# Autodesk Inventor assembly: electromag_gimbal
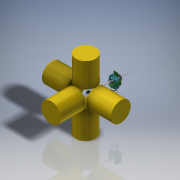
[picture p0: Inventor's stored thumbnail of the model, 180x180]
Saved by Autodesk Inventor 2019 (Build 230136000, 136)
## iProperties
Created: 2018-08-27
Part Number: electromag_gimbal
Document SubType Name: Assembly
Designer: Brian
Author: Brian
## Documents named in this file (13)
- C:\Users\Brian\Desktop\designs\gimbal\electromag_gimbal.iam
- C:\Users\Brian\Desktop\designs\gimbal\aluminum rod.ipt
- C:\Users\Brian\Desktop\designs\gimbal\61205K720_FIXED ALIGNMENT LINEAR BALL BRNG.ipt
- C:\Users\Brian\Desktop\designs\gimbal\magnet.ipt
- C:\Users\Brian\Desktop\designs\gimbal\angle hall sensor.ipt
- C:\Users\Brian\Desktop\designs\gimbal\top_g2.ipt
- C:\Users\Brian\Desktop\designs\gimbal\bottom_g2v2.ipt
- C:\Users\Brian\Desktop\designs\gimbal\RS05P8E-Step.ipt
- C:\Users\Brian\Desktop\designs\gimbal\shaft_hall_mount.ipt
- C:\Users\Brian\Desktop\designs\gimbal\magnet_stop.ipt
- C:\Users\Brian\Desktop\designs\gimbal\end_stop.ipt
- C:\Users\Brian\Desktop\designs\gimbal\electromagnet.ipt
- C:\Users\Brian\Desktop\designs\gimbal\eye_nut_scaled_more.ipt
## Components (18 placed, 12 different names)
1. aluminum rod:1 — Mate:2, Mate:3, Tangent:1, Tangent:2, Mate:21, Mate:26, Mate:29, Mate:30, Flush:5
2. 61205K720_FIXED ALIGNMENT LINEAR BALL BRNG:1 — Mate:2, Mate:5, Flush:4, Mate:16
3. magnet:1 — Mate:3, Tangent:1, Tangent:2, Mate:5, Flush:2
4. angle hall sensor:1 — Mate:19, Mate:24, Mate:25
5. angle hall sensor:2 — Mate:6, Mate:7, Mate:8, Flush:2
6. angle hall sensor:3 — Mate:9, Mate:10, Mate:11
7. top_g2:1 — Mate:6, Mate:7, Mate:8, Mate:9, Mate:10, Mate:11, Mate:12, Flush:3, Mate:13, Mate:17, Mate:18, Mate:23
8. bottom_g2v2:1 — Mate:12, Flush:3, Mate:13, Mate:14, Mate:15
9. RS05P8E-Step:1 — Mate:14, Mate:15
10. shaft_hall_mount:1 — Flush:4, Mate:16, Mate:17, Mate:18, Mate:19, Mate:24, Mate:25, Mate:28
11. magnet_stop:1 — Mate:21, Mate:23, Mate:27, Flush:5
12. end_stop:1 — Mate:26, Mate:27, Mate:28
13. electromagnet:1
14. electromagnet:2
15. electromagnet:3
16. electromagnet:4
17. electromagnet:5
18. eye_nut_scaled_more:1 — Mate:29, Mate:30
## Relationships (32: Mate 26, Flush 4, Tangent 2)
- Mate:2: aluminum rod:1 ↔ 61205K720_FIXED ALIGNMENT LINEAR BALL BRNG:1
- Mate:3: aluminum rod:1 ↔ magnet:1
- Tangent:1 (-7 mm): aluminum rod:1 ↔ magnet:1
- Tangent:2 (-7 mm): aluminum rod:1 ↔ magnet:1
- Mate:5: 61205K720_FIXED ALIGNMENT LINEAR BALL BRNG:1 ↔ magnet:1
- Mate:6 (6 mm): angle hall sensor:2 ↔ top_g2:1
- Mate:7: angle hall sensor:2 ↔ top_g2:1
- Mate:8: angle hall sensor:2 ↔ top_g2:1
- Flush:2: magnet:1 ↔ angle hall sensor:2
- Mate:9 (7 mm): angle hall sensor:3 ↔ top_g2:1
- Mate:10: angle hall sensor:3 ↔ top_g2:1
- Mate:11: angle hall sensor:3 ↔ top_g2:1
- Mate:12 (1 mm): top_g2:1 ↔ bottom_g2v2:1
- Flush:3: top_g2:1 ↔ bottom_g2v2:1
- Mate:13: top_g2:1 ↔ bottom_g2v2:1
- Mate:14 (2 mm): bottom_g2v2:1 ↔ RS05P8E-Step:1
- Mate:15: bottom_g2v2:1 ↔ RS05P8E-Step:1
- Flush:4 (-1 mm): 61205K720_FIXED ALIGNMENT LINEAR BALL BRNG:1 ↔ shaft_hall_mount:1
- Mate:16: 61205K720_FIXED ALIGNMENT LINEAR BALL BRNG:1 ↔ shaft_hall_mount:1
- Mate:17 (2 mm): top_g2:1 ↔ shaft_hall_mount:1
- Mate:18: top_g2:1 ↔ shaft_hall_mount:1
- Mate:19: angle hall sensor:1 ↔ shaft_hall_mount:1
- Mate:21: aluminum rod:1 ↔ magnet_stop:1
- Mate:23: top_g2:1 ↔ magnet_stop:1
- Mate:24: angle hall sensor:1 ↔ shaft_hall_mount:1
- Mate:25: angle hall sensor:1 ↔ shaft_hall_mount:1
- Mate:26: aluminum rod:1 ↔ end_stop:1
- Mate:27 (44.45 mm): magnet_stop:1 ↔ end_stop:1
- Mate:28: shaft_hall_mount:1 ↔ end_stop:1
- Mate:29: aluminum rod:1 ↔ eye_nut_scaled_more:1
- Mate:30: aluminum rod:1 ↔ eye_nut_scaled_more:1
- Flush:5 (55.88 mm): aluminum rod:1 ↔ magnet_stop:1
